# Autodesk Inventor assembly: Assembly1
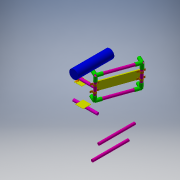
[picture p0: Inventor's stored thumbnail of the model, 180x180]
Saved by Autodesk Inventor 2016 (Build 200138000, 138)
## iProperties
Created: 2017-01-30
Part Number: Assembly1
Document SubType Name: Assembly
Designer: student1
Author: student1
## Documents named in this file (8)
- C:\Users\student1\Desktop\Python code\CAD\ROV\OldVersions\Assembly1.iam
- C:\Users\student1\Desktop\Python code\CAD\ROV\Control Pipe.ipt
- C:\Users\student1\Desktop\Python code\CAD\ROV\Frame Part 1.ipt
- C:\Users\student1\Desktop\Python code\CAD\ROV\Attachy-thing.ipt
- C:\Users\student1\Desktop\Python code\CAD\ROV\Control pipe holder.ipt
- C:\Users\student1\Desktop\Python code\CAD\ROV\motor holder.ipt
- C:\Users\student1\Desktop\Python code\CAD\ROV\pvc 1in 3 way elbow noah.ipt
- C:\Users\student1\Desktop\Python code\CAD\ROV\Frame Part 1.5.ipt
## Components (22 placed, 7 different names)
1. Control Pipe:1
2. Frame Part 1:1 — Mate:1, Mate:2, Mate:5, Mate:6, Mate:37, Mate:38, Mate:39, Mate:40
3. Frame Part 1:2 — Mate:3, Mate:4, Mate:7, Mate:8, Mate:9, Mate:10, Mate:33, Mate:34, Mate:35, Mate:36
4. Attachy-thing:1 — Mate:3, Mate:7, Mate:8, Mate:11, Mate:16
5. Attachy-thing:2 — Mate:4, Mate:9, Mate:10, Mate:12, Mate:14
6. Attachy-thing:3 — Mate:1, Mate:6, Mate:18, Mate:21
7. Attachy-thing:4 — Mate:2, Mate:5, Mate:17, Mate:19
8. Control pipe holder:1 — Mate:11, Mate:12, Mate:14, Mate:16, Mate:17, Mate:18, Mate:19, Mate:21
9. Frame Part 1:3 — Mate:29, Mate:30
10. Frame Part 1:4 — Mate:27, Mate:28
11. Attachy-thing:5 — Mate:23, Mate:24, Mate:27, Mate:28, Mate:31
12. Attachy-thing:7 — Mate:25, Mate:26, Mate:29, Mate:30, Mate:32
13. motor holder:1 — Mate:25, Mate:26, Mate:32
14. motor holder:2 — Mate:23, Mate:24, Mate:31
15. pvc 1in 3 way elbow noah:1 — Mate:35, Mate:36, Mate:42, Mate:43
16. pvc 1in 3 way elbow noah:2 — Mate:33, Mate:34, Mate:44, Mate:46
17. pvc 1in 3 way elbow noah:3 — Mate:38, Mate:39, Mate:41, Mate:48
18. pvc 1in 3 way elbow noah:4 — Mate:37, Mate:40, Mate:45, Mate:47
19. Frame Part 1.5:1 — Mate:44, Mate:45, Mate:46, Mate:47
20. Frame Part 1.5:2 — Mate:41, Mate:42, Mate:43, Mate:48
21. Frame Part 1.5:3
22. Frame Part 1.5:4
## Relationships (44: Mate 44)
- Mate:1: Frame Part 1:1 ↔ Attachy-thing:3
- Mate:2: Frame Part 1:1 ↔ Attachy-thing:4
- Mate:3: Frame Part 1:2 ↔ Attachy-thing:1
- Mate:4: Frame Part 1:2 ↔ Attachy-thing:2
- Mate:5: Frame Part 1:1 ↔ Attachy-thing:4
- Mate:6: Frame Part 1:1 ↔ Attachy-thing:3
- Mate:7: Frame Part 1:2 ↔ Attachy-thing:1
- Mate:8: Frame Part 1:2 ↔ Attachy-thing:1
- Mate:9: Frame Part 1:2 ↔ Attachy-thing:2
- Mate:10: Frame Part 1:2 ↔ Attachy-thing:2
- Mate:11: Attachy-thing:1 ↔ Control pipe holder:1
- Mate:12: Attachy-thing:2 ↔ Control pipe holder:1
- Mate:14: Attachy-thing:2 ↔ Control pipe holder:1
- Mate:16: Attachy-thing:1 ↔ Control pipe holder:1
- Mate:17: Attachy-thing:4 ↔ Control pipe holder:1
- Mate:18: Attachy-thing:3 ↔ Control pipe holder:1
- Mate:19: Attachy-thing:4 ↔ Control pipe holder:1
- Mate:21: Attachy-thing:3 ↔ Control pipe holder:1
- Mate:23: Attachy-thing:5 ↔ motor holder:2
- Mate:24: Attachy-thing:5 ↔ motor holder:2
- Mate:25: Attachy-thing:7 ↔ motor holder:1
- Mate:26: Attachy-thing:7 ↔ motor holder:1
- Mate:27: Frame Part 1:4 ↔ Attachy-thing:5
- Mate:28: Frame Part 1:4 ↔ Attachy-thing:5
- Mate:29: Frame Part 1:3 ↔ Attachy-thing:7
- Mate:30: Frame Part 1:3 ↔ Attachy-thing:7
- Mate:31: Attachy-thing:5 ↔ motor holder:2
- Mate:32: Attachy-thing:7 ↔ motor holder:1
- Mate:33: Frame Part 1:2 ↔ pvc 1in 3 way elbow noah:2
- Mate:34: Frame Part 1:2 ↔ pvc 1in 3 way elbow noah:2
- Mate:35: Frame Part 1:2 ↔ pvc 1in 3 way elbow noah:1
- Mate:36: Frame Part 1:2 ↔ pvc 1in 3 way elbow noah:1
- Mate:37: Frame Part 1:1 ↔ pvc 1in 3 way elbow noah:4
- Mate:38: Frame Part 1:1 ↔ pvc 1in 3 way elbow noah:3
- Mate:39: Frame Part 1:1 ↔ pvc 1in 3 way elbow noah:3
- Mate:40: Frame Part 1:1 ↔ pvc 1in 3 way elbow noah:4
- Mate:41: pvc 1in 3 way elbow noah:3 ↔ Frame Part 1.5:2
- Mate:42: pvc 1in 3 way elbow noah:1 ↔ Frame Part 1.5:2
- Mate:43: pvc 1in 3 way elbow noah:1 ↔ Frame Part 1.5:2
- Mate:44: pvc 1in 3 way elbow noah:2 ↔ Frame Part 1.5:1
- Mate:45: pvc 1in 3 way elbow noah:4 ↔ Frame Part 1.5:1
- Mate:46: pvc 1in 3 way elbow noah:2 ↔ Frame Part 1.5:1
- Mate:47: pvc 1in 3 way elbow noah:4 ↔ Frame Part 1.5:1
- Mate:48: pvc 1in 3 way elbow noah:3 ↔ Frame Part 1.5:2
